# Autodesk Inventor assembly: Grabber with Stamp
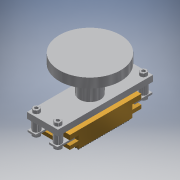
[picture p0: Inventor's stored thumbnail of the model, 180x180]
Saved by Autodesk Inventor 2019.4 (Build 234330000, 330)
## iProperties
Created: 2021-01-07
Part Number: Grabber with Stamp
Document SubType Name: Assembly
Designer: caleb
Author: caleb
## Documents named in this file (3)
- C:\Users\cfang\Desktop\nebraska-silicon-lab\CAD\ETL\Module Assembly\Grabber with Stamp.iam
- C:\Users\cfang\Desktop\nebraska-silicon-lab\CAD\ETL\Module Assembly\Grabber Tool\Grabber Tool.iam
- C:\Users\cfang\Desktop\nebraska-silicon-lab\CAD\ETL\Module Assembly\Glue Stamp\Stamp Assembly.iam
## Components (2 placed, 2 different names)
1. Grabber Tool:1 [sub-assembly] — Mate:1, Angle:1
2. Stamp Assembly:1 [sub-assembly] — Mate:1, Angle:1
## Relationships (2: Mate 1, Angle 1)
- Mate:1: Grabber Tool:1 ↔ Stamp Assembly:1
- Angle:1 (0 deg): Grabber Tool:1 ↔ Stamp Assembly:1
